# Autodesk Inventor assembly: 5 pin header
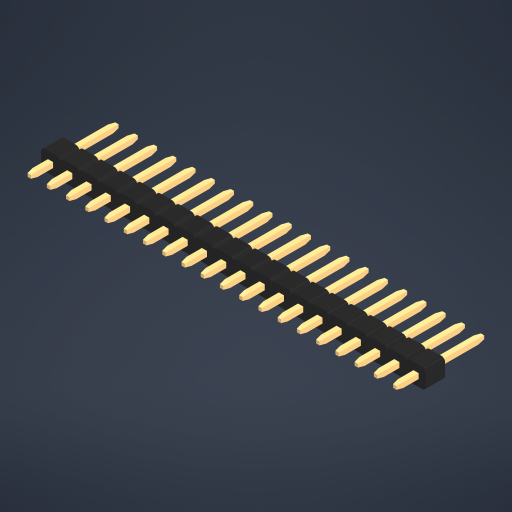
[picture p0: Inventor's stored thumbnail of the model, 512x512]
Saved by Autodesk Inventor 2024 (Build 280153000, 153)
## iProperties
Created: 2025-11-30
Part Number: 5 pin header
Document SubType Name: Assembly
Designer: Vincent Larson
Author: Vincent Larson
## Documents named in this file (3)
- C:\Users\Vincent Larson\Downloads\Digital Ship Challenge\Digital Ship Challenge Remote\Pin Headers\5 pin header.iam
- C:\Users\Vincent Larson\Downloads\Digital Ship Challenge\Digital Ship Challenge Remote\Pin Headers\spacer.ipt
- C:\Users\Vincent Larson\Downloads\Digital Ship Challenge\Digital Ship Challenge Remote\Pin Headers\pins.ipt
## Components (2 placed, 2 different names)
1. spacer_2 — Mate:1, Mate:2
2. pins 1-20_5 — Mate:1, Mate:2
## Relationships (2: Mate 2)
- Mate:1: spacer_2 ↔ pins 1-20_5
- Mate:2: spacer_2 ↔ pins 1-20_5
